# Autodesk Inventor assembly: az_rot_mot_asm.ipt
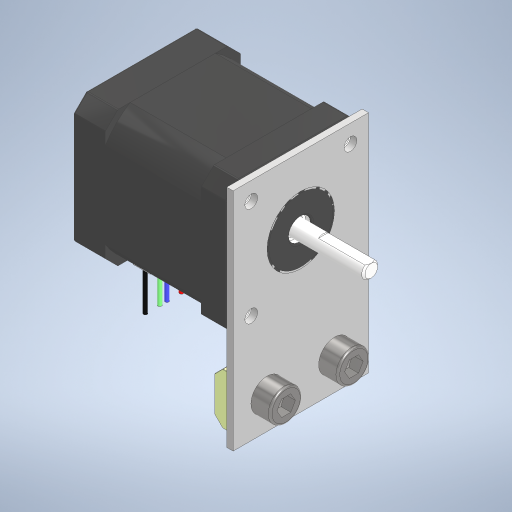
[picture p0: Inventor's stored thumbnail of the model, 512x512]
Saved by Autodesk Inventor 2024 (Build 280153000, 153)
## iProperties
Created: 2025-12-18
Part Number: az_rot_mot_asm.ipt
Document SubType Name: Assembly
Designer: schar
Author: schar
## Documents named in this file (6)
- C:\Users\schar\Desktop\projectBlueprint\AMSTS\hardware\az_rot_mot_asm.ipt.iam
- C:\Users\schar\Desktop\projectBlueprint\AMSTS\hardware\az_rot_mot_holder.iam.ipt
- C:\Users\schar\Desktop\projectBlueprint\AMSTS\hardware\17HE19-2004S.ipt
- C:\Users\schar\Documents\Inventor\Content Center Files\R2024\en-US\ISO 4762(1)\DIN EN ISO 4762 - M6 x 10.ipt
- C:\Users\schar\Desktop\projectBlueprint\AMSTS\hardware\3030_tnut_m6_MIR_MIR.ipt
- az_rot_mot_holder.iam
## Components (6 placed, 4 different names)
1. az_rot_mot_holder.iam:1 — Mate:1, Mate:2, Mate:3, Mate:4, Mate:5, Mate:6, Mate:7, Mate:9, Mate:11
2. 17HE19-2004S:1 — Mate:1, Mate:2, Mate:3
3. DIN EN ISO 4762 M6 x 10:1 — Mate:4, Mate:6, Mate:8
4. DIN EN ISO 4762 M6 x 10:2 — Mate:5, Mate:7, Mate:10
5. 3030_tnut_m6_MIR_MIR:1 — Mate:10, Mate:11
6. 3030_tnut_m6_MIR_MIR:2 — Mate:8, Mate:9
## Relationships (11: Mate 11)
- Mate:1: az_rot_mot_holder.iam:1 ↔ 17HE19-2004S:1
- Mate:2: az_rot_mot_holder.iam:1 ↔ 17HE19-2004S:1
- Mate:3: az_rot_mot_holder.iam:1 ↔ 17HE19-2004S:1
- Mate:4: az_rot_mot_holder.iam:1 ↔ DIN EN ISO 4762 M6 x 10:1
- Mate:5: az_rot_mot_holder.iam:1 ↔ DIN EN ISO 4762 M6 x 10:2
- Mate:6: az_rot_mot_holder.iam:1 ↔ DIN EN ISO 4762 M6 x 10:1
- Mate:7: az_rot_mot_holder.iam:1 ↔ DIN EN ISO 4762 M6 x 10:2
- Mate:8: DIN EN ISO 4762 M6 x 10:1 ↔ 3030_tnut_m6_MIR_MIR:2
- Mate:9 (0.357 mm): az_rot_mot_holder.iam:1 ↔ 3030_tnut_m6_MIR_MIR:2
- Mate:10: DIN EN ISO 4762 M6 x 10:2 ↔ 3030_tnut_m6_MIR_MIR:1
- Mate:11 (0.357 mm): az_rot_mot_holder.iam:1 ↔ 3030_tnut_m6_MIR_MIR:1
